# Autodesk Inventor assembly: Functioning swerve drive (casing)
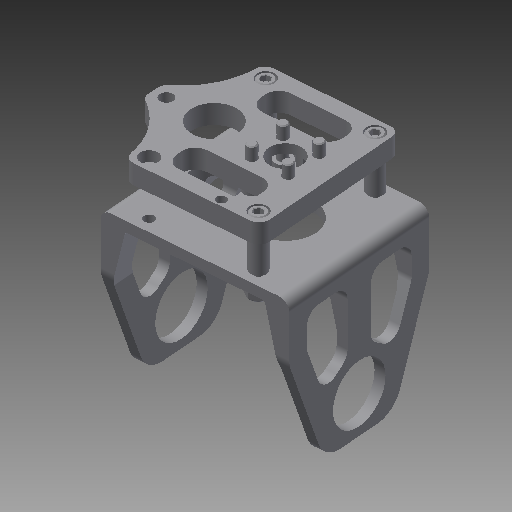
[picture p0: Inventor's stored thumbnail of the model, 512x512]
Saved by Autodesk Inventor 2019 (Build 230136000, 136)
## iProperties
Created: 2019-01-14
Part Number: Functioning swerve drive (casing)
Document SubType Name: Assembly
Designer: josh
Mass: 99.698 g
Surface Area: 507.638 cm^2
Volume: 99.698 cm^3
Density: 1 g/cm^3
Author: josh
## Documents named in this file (7)
- D:\Synthesis Robots\Epsilon\Functioning swerve drive sub-assemblies\Functioning swerve drive (casing).iam
- D:\Synthesis Robots\Epsilon\Swerve drive parts\AMS C Housing Rev 2.ipt
- D:\Synthesis Robots\Epsilon\Swerve drive parts\10-32 Nylock Nut 1_90631A411.ipt
- D:\Synthesis Robots\Epsilon\Swerve drive parts\10-32x1250_shcs.ipt
- D:\Synthesis Robots\Epsilon\Swerve drive parts\620x215 alum spacer 83062 K-S.ipt
- D:\Synthesis Robots\Epsilon\Swerve drive parts\Gear Plate.ipt
- D:\Synthesis Robots\Epsilon\Swerve drive parts\10-32x0625_shcs_HX-SHCS 0.19-32x1.375x1-C.ipt
## Components (15 placed, 6 different names)
1. AMS C Housing Rev 2:1
2. 10-32 Nylock Nut 1_90631A411:1
3. 10-32 Nylock Nut 1_90631A411:2
4. 10-32 Nylock Nut 1_90631A411:3
5. 10-32x1250_shcs:1
6. 10-32x1250_shcs:2
7. 10-32x1250_shcs:3
8. 620x215 alum spacer 83062 K-S:1
9. 620x215 alum spacer 83062 K-S:2
10. 620x215 alum spacer 83062 K-S:3
11. 10-32x0625_shcs_HX-SHCS 0.19-32x1.375x1-C:1
12. 10-32x0625_shcs_HX-SHCS 0.19-32x1.375x1-C:2
13. 10-32x0625_shcs_HX-SHCS 0.19-32x1.375x1-C:3
14. 10-32x0625_shcs_HX-SHCS 0.19-32x1.375x1-C:4
15. Gear Plate:1
## Relationships (20: Mate 14, RevoluteJoint 3, Flush 3)
- [RevoluteJoint]: 10-32 Nylock Nut 1_90631A411:1 ↔ 10-32x1250_shcs:3
- [RevoluteJoint]: 10-32 Nylock Nut 1_90631A411:3 ↔ 10-32x1250_shcs:2
- [RevoluteJoint]: 10-32 Nylock Nut 1_90631A411:2 ↔ 10-32x1250_shcs:1
- [Mate]: 10-32x1250_shcs:2 ↔ Gear Plate:1
- [Mate]: 10-32x1250_shcs:2 ↔ 620x215 alum spacer 83062 K-S:2
- [Flush]: 10-32x1250_shcs:2 ↔ Gear Plate:1
- [Mate]: 620x215 alum spacer 83062 K-S:2 ↔ Gear Plate:1
- [Mate]: 10-32x1250_shcs:1 ↔ Gear Plate:1
- [Mate]: 10-32x1250_shcs:1 ↔ 620x215 alum spacer 83062 K-S:1
- [Flush]: 10-32x1250_shcs:1 ↔ Gear Plate:1
- [Mate]: 620x215 alum spacer 83062 K-S:1 ↔ Gear Plate:1
- [Mate]: 10-32x1250_shcs:3 ↔ 620x215 alum spacer 83062 K-S:3
- [Flush]: 10-32x1250_shcs:3 ↔ Gear Plate:1
- [Mate]: 10-32x1250_shcs:3 ↔ Gear Plate:1
- [Mate]: 620x215 alum spacer 83062 K-S:3 ↔ Gear Plate:1
- [Mate]: AMS C Housing Rev 2:1 ↔ 10-32x1250_shcs:2
- [Mate]: AMS C Housing Rev 2:1 ↔ 10-32x1250_shcs:1
- [Mate]: 10-32x0625_shcs_HX-SHCS 0.19-32x1.375x1-C:4 ↔ Gear Plate:1
- [Mate]: 10-32x0625_shcs_HX-SHCS 0.19-32x1.375x1-C:2 ↔ Gear Plate:1
- [Mate]: 10-32x0625_shcs_HX-SHCS 0.19-32x1.375x1-C:1 ↔ Gear Plate:1
## Named parameters: d398_d207 = 0 mm, d399_d209 = 0 mm, d287_d94_d139 = 0 mm, d288_d95_d140 = -154.263513 deg, d289_d96_d141 = 0 mm, d290_d97_d142 = 63.496867 deg, d291_d98_d143 = 0 mm, d292_d99_d144 = 150.286815 deg, d293_d100_d146 = 0 mm, d294_d101_d147 = 0 mm, d295_d102_d148 = 0 mm, d296_d103_d149 = 0 mm, d297_d104_d150 = 0 mm, d298_d122_d151 = 0 mm, d299_d123_d152 = 0 mm, d300_d124_d153 = 0 mm, d305_d129_d158 = 0 mm, d306_d130_d159 = 0 mm, d307_d131_d160 = 0 mm, d308_d132_d161 = 0 mm
